# Autodesk Inventor assembly: ElectronicsBatteryAssembly
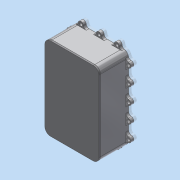
[picture p0: Inventor's stored thumbnail of the model, 180x180]
Saved by Autodesk Inventor 2017 (Build 210142000, 142)
## iProperties
Created: 2018-02-14
Part Number: ElectronicsBatteryAssembly
Document SubType Name: Assembly
Designer: Derek Wider
Author: Derek Wider
## Documents named in this file (8)
- G:\Projects\Submarine\Submarine-project\CAD\common\ElectronicsBatteryAssembly.iam
- G:\Projects\Submarine\Submarine-project\CAD\common\ElectronicsBatteryNoConnector.ipt
- G:\Projects\Submarine\Submarine-project\CAD\common\Connectors\XT60\XT60 Connector Female Connector.iam
- G:\Projects\Submarine\Submarine-project\CAD\fore\BatteryCaseSide1.ipt
- G:\Projects\Submarine\Submarine-project\CAD\fore\BatteryCaseSide2.ipt
- G:\Projects\Submarine\Submarine-project\CAD\fore\BatteryCaseORing.ipt
- G:\Projects\Submarine\Submarine-project\CAD\fore\BatteryCaseSide3.ipt
- G:\Projects\Submarine\Submarine-project\CAD\common\ThreadedRod_Nuts_Bolts\Bolt_SocketHead_Hex_Thread_5_40_7_16length.ipt
## Components (7 placed, 7 different names)
1. ElectronicsBatteryNoConnector:1 — Mate:1, Mate:2, Angle:1, Mate:6, Mate:7, Mate:8
2. XT60 Connector Female Connector:1 [sub-assembly] — Mate:1, Mate:2, Angle:1
3. BatteryCaseSide1:1 — Tangent:1, Tangent:2, Tangent:3, Tangent:4, Mate:5, Flush:1, Flush:2, Mate:7, Mate:8, Mate:9, Flush:3, Flush:4, Mate:10, Mate:11
4. BatteryCaseSide2:1 — Mate:9, Flush:3, Flush:4
5. BatteryCaseORing:1 — Tangent:1, Tangent:2, Tangent:3, Tangent:4
6. BatteryCaseSide3:1 — Mate:5, Flush:1, Flush:2, Mate:6
7. Bolt_SocketHead_Hex_Thread_5_40_7_16length:1 — Mate:10, Mate:11
## Relationships (18: Mate 9, Tangent 4, Flush 4, Angle 1)
- Mate:1: ElectronicsBatteryNoConnector:1 ↔ XT60 Connector Female Connector:1
- Mate:2: ElectronicsBatteryNoConnector:1 ↔ XT60 Connector Female Connector:1
- Angle:1 (0 deg): ElectronicsBatteryNoConnector:1 ↔ XT60 Connector Female Connector:1
- Tangent:1: BatteryCaseSide1:1 ↔ BatteryCaseORing:1
- Tangent:2: BatteryCaseSide1:1 ↔ BatteryCaseORing:1
- Tangent:3 (1.27 mm): BatteryCaseSide1:1 ↔ BatteryCaseORing:1
- Tangent:4 (1.27 mm): BatteryCaseSide1:1 ↔ BatteryCaseORing:1
- Mate:5: BatteryCaseSide1:1 ↔ BatteryCaseSide3:1
- Flush:1: BatteryCaseSide1:1 ↔ BatteryCaseSide3:1
- Flush:2: BatteryCaseSide1:1 ↔ BatteryCaseSide3:1
- Mate:6: ElectronicsBatteryNoConnector:1 ↔ BatteryCaseSide3:1
- Mate:7 (6.35 mm): ElectronicsBatteryNoConnector:1 ↔ BatteryCaseSide1:1
- Mate:8 (6.35 mm): ElectronicsBatteryNoConnector:1 ↔ BatteryCaseSide1:1
- Mate:9: BatteryCaseSide1:1 ↔ BatteryCaseSide2:1
- Flush:3: BatteryCaseSide1:1 ↔ BatteryCaseSide2:1
- Flush:4: BatteryCaseSide1:1 ↔ BatteryCaseSide2:1
- Mate:10: BatteryCaseSide1:1 ↔ Bolt_SocketHead_Hex_Thread_5_40_7_16length:1
- Mate:11: BatteryCaseSide1:1 ↔ Bolt_SocketHead_Hex_Thread_5_40_7_16length:1
